# Autodesk Inventor assembly: Soporte v2
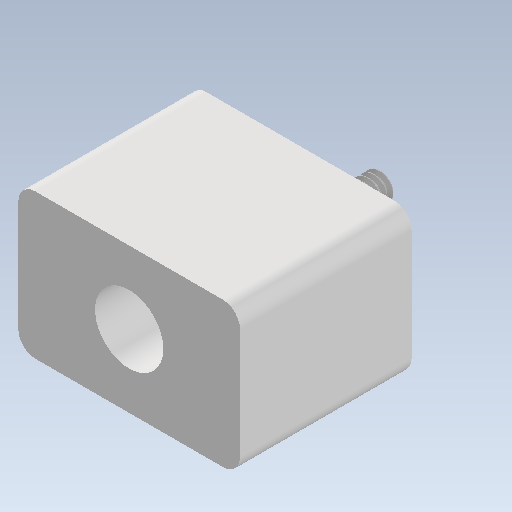
[picture p0: Inventor's stored thumbnail of the model, 512x512]
Saved by Autodesk Inventor 2020.3 (Build 243373000, 373)
## iProperties
Created: 2020-06-15
Part Number: Soporte v2
Document SubType Name: Assembly
Designer: javic
Author: javic
## Documents named in this file (4)
- C:\Users\javic\Downloads\Universidad\2020-1\Seminario - SPEL\InterStage\Componentes\Piezas\Soporte v2.iam
- C:\Users\javic\Downloads\Universidad\2020-1\Seminario - SPEL\InterStage\Componentes\Piezas\Soporte v2.ipt
- C:\Users\javic\Downloads\Universidad\2020-1\Seminario - SPEL\InterStage\Componentes\Piezas\Golilla M1.6  .ipt
- C:\Users\javic\Downloads\Universidad\2020-1\Seminario - SPEL\InterStage\Componentes\Piezas\Tornillo M1.6 8 mm.ipt
## Components (3 placed, 3 different names)
1. Soporte v2:1 — Coincidencia:1, Coincidencia:2, Coincidencia:3
2. Golilla M1.6  :1 — Coincidencia:1, Coincidencia:2, Coincidencia:4
3. Tornillo M1.6 8 mm:1 — Coincidencia:3, Coincidencia:4
## Relationships (4: Mate 4)
- Coincidencia:1 [Mate]: Soporte v2:1 ↔ Golilla M1.6  :1
- Coincidencia:2 [Mate]: Soporte v2:1 ↔ Golilla M1.6  :1
- Coincidencia:3 [Mate]: Soporte v2:1 ↔ Tornillo M1.6 8 mm:1
- Coincidencia:4 [Mate]: Golilla M1.6  :1 ↔ Tornillo M1.6 8 mm:1
